# Autodesk Inventor assembly: canaletaInferior
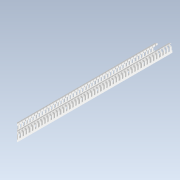
[picture p0: Inventor's stored thumbnail of the model, 180x180]
Saved by Autodesk Inventor 2021 (Build 250183000, 183)
## iProperties
Created: 2021-07-05
Part Number: canaletaInferior
Document SubType Name: Assembly
Designer: Andrés Holguín
Author: Andrés Holguín
## Documents named in this file (2)
- C:\Users\andre\Downloads\Diseño mecatrónico\Parcial 2\Cad\Canaletas\canaletaInferior.iam
- C:\Users\andre\Downloads\Diseño mecatrónico\Parcial 2\Cad\Canaletas\7308-1.iam
## Components (5 placed, 1 different names)
1. 7308-1:1 [sub-assembly] — Rigid:1, Mate:2, Angle:2
2. 7308-1:2 [sub-assembly] — Rigid:1, Rigid:2
3. 7308-1:3 [sub-assembly] — Rigid:2, Rigid:3
4. 7308-1:4 [sub-assembly] — Rigid:3, Rigid:4
5. 7308-1:5 [sub-assembly] — Rigid:4, Mate:1, Angle:1
## Relationships (8: WeldJoint 4, Mate 2, Angle 2)
- Rigid:1 [WeldJoint]: 7308-1:1 ↔ 7308-1:2
- Rigid:2 [WeldJoint]: 7308-1:2 ↔ 7308-1:3
- Rigid:3 [WeldJoint]: 7308-1:3 ↔ 7308-1:4
- Rigid:4 [WeldJoint]: 7308-1:4 ↔ 7308-1:5
- Mate:1: 7308-1:5
- Angle:1 (45 deg): 7308-1:5
- Mate:2: 7308-1:1
- Angle:2 (45 deg): 7308-1:1
